# Autodesk Inventor assembly: CribbageBoardAssembly
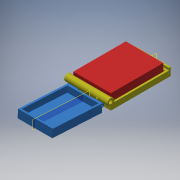
[picture p0: Inventor's stored thumbnail of the model, 180x180]
Saved by Autodesk Inventor 2017 SP1 (Build 210196100, 196)
## iProperties
Created: 2016-10-19
Part Number: CribbageBoardAssembly
Document SubType Name: Assembly
Designer: steele
Author: steele
## Documents named in this file (4)
- D:\snobotics\CAD-Development\robSteele\HouseProjects\CribbageBoard\CribbageBoardAssembly.iam
- D:\snobotics\CAD-Development\robSteele\HouseProjects\CribbageBoard\BottomHalfOfBoard.ipt
- D:\snobotics\CAD-Development\robSteele\HouseProjects\CribbageBoard\CardDeck.ipt
- D:\snobotics\CAD-Development\robSteele\HouseProjects\CribbageBoard\TopHalfOfBoard.ipt
## Components (3 placed, 3 different names)
1. BottomHalfOfBoard:1 — Mate:1, Mate:2, Mate:3, Flush:1
2. CardDeck:1 — Mate:1, Mate:2, Mate:3
3. TopHalfOfBoard:1 — Flush:1
## Relationships (4: Mate 3, Flush 1)
- Mate:1: BottomHalfOfBoard:1 ↔ CardDeck:1
- Mate:2: BottomHalfOfBoard:1 ↔ CardDeck:1
- Mate:3: BottomHalfOfBoard:1 ↔ CardDeck:1
- Flush:1: BottomHalfOfBoard:1 ↔ TopHalfOfBoard:1
## Named parameters: cardDeckWidth = 50.8 mm, cardDeckLength = 76.2 mm, cardDeckDepth = 14.2875 mm, materialWallThickness = 3.175 mm, baseWallThickness = 3.175 mm
